# Autodesk Inventor assembly: ASY ДМФ 0100 Барабан v2.1
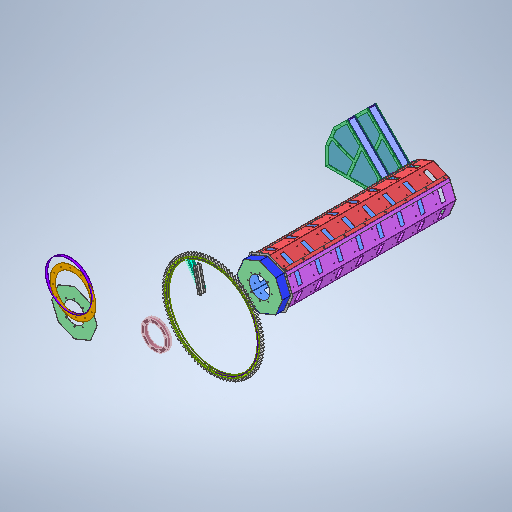
[picture p0: Inventor's stored thumbnail of the model, 512x512]
Saved by Autodesk Inventor 2025 (Build 290162010, 162A)
## iProperties
Created: 2024-04-28
Part Number: ASY ДМФ 0100 Барабан v2.1
Document SubType Name: Assembly
Designer: pokla
Author: pokla
## Documents named in this file (25)
- C:\Users\pokla\Documents\Inventor\ДФО\ДМФ\DMF-Disk-Micro-Filter\Барабан v2.1\ASY ДМФ 0100 Барабан v2.1.iam
- C:\Users\pokla\Documents\Inventor\ДФО\ДМФ\DMF-Disk-Micro-Filter\Барабан v2.1\DMF 01 21 Барабан торец НОС v2.1.ipt
- C:\Users\pokla\Documents\Inventor\ДФО\ДМФ\DMF-Disk-Micro-Filter\Барабан v2.1\DMF 01 13 Барабан Лист лев брт v2.1.ipt
- C:\Users\pokla\Documents\Inventor\ДФО\ДМФ\DMF-Disk-Micro-Filter\Барабан v2.1\DMF 01 14 Барабан Лист прав брт v2.1.ipt
- C:\Users\pokla\Documents\Inventor\ДФО\ДМФ\DMF-Disk-Micro-Filter\Барабан v2.1\DMF 01 31 Барабан Опорное кольцо НОС v2.1.ipt
- C:\Users\pokla\Documents\Inventor\ДФО\ДМФ\DMF-Disk-Micro-Filter\Барабан v2.1\DMF 01 17 опора крышки v2.1.ipt
- C:\Users\pokla\Documents\Inventor\ДФО\ДМФ\DMF-Disk-Micro-Filter\Барабан v2.1\DMF 000 размеры v2.1.ipt
- C:\Users\pokla\Documents\Inventor\ДФО\ДМФ\DMF-Disk-Micro-Filter\Барабан v2.1\DMF 01 12 Барабан усилитель v2.1.ipt
- C:\Users\pokla\Documents\Inventor\ДФО\ДМФ\DMF-Disk-Micro-Filter\Барабан v2.1\ASY DMF 010 cap v2.1.iam
- C:\Users\pokla\Documents\Inventor\ДФО\ДМФ\DMF-Disk-Micro-Filter\Барабан v2.1\DMF 01 32 Барабан Опорное кольцо КОРМА v2.1.ipt
- C:\Users\pokla\Documents\Inventor\ДФО\ДМФ\DMF-Disk-Micro-Filter\Барабан v2.1\DMF 01 22 Барабан торец КОРМА v2.1.ipt
- C:\Users\pokla\Documents\Inventor\ДФО\ДМФ\DMF-Disk-Micro-Filter\Барабан v2.1\ASY DMF filter package v2.1.iam
- C:\Users\pokla\Documents\Inventor\ДФО\ДМФ\DMF-Disk-Micro-Filter\Барабан v2.1\DMF 01 21 cylinder butt end nose.ipt
- C:\Users\pokla\Documents\Inventor\ДФО\ДМФ\DMF-Disk-Micro-Filter\Барабан v2.1\DMF 2.1 01 42 Gear way 2.ipt
- C:\Users\pokla\Documents\Inventor\ДФО\ДМФ\DMF-Disk-Micro-Filter\Барабан v2.1\DMF 2.1 01 43 Gear rim 3.ipt
- C:\Users\pokla\Documents\Inventor\ДФО\ДМФ\DMF-Disk-Micro-Filter\Барабан v2.1\DMF 2.1 01 44 Gear rim 4.ipt
- C:\Users\pokla\Documents\Inventor\ДФО\ДМФ\DMF-Disk-Micro-Filter\Барабан v2.1\DMF 2.1 01 45 Gear ring 5.ipt
- C:\Users\pokla\Documents\Inventor\ДФО\ДМФ\DMF-Disk-Micro-Filter\Барабан v2.1\DMF 2.1 01 46 Gear axis wheel 6.ipt
- C:\Users\pokla\Documents\Inventor\ДФО\ДМФ\DMF-Disk-Micro-Filter\Барабан v2.1\DMF 01 13 Барабан усилитель v2.1.ipt
- C:\Users\pokla\Documents\Inventor\ДФО\ДМФ\DMF-Disk-Micro-Filter\шестерни 06.09.2025\DMF sector big gear 2.1.ipt
- C:\Users\pokla\Documents\Inventor\ДФО\ДМФ\DMF-Disk-Micro-Filter\Барабан v2.1\DMF 01 15 drum sheet 1.ipt
- C:\Users\pokla\Documents\Inventor\ДФО\ДМФ\DMF-Disk-Micro-Filter\ДМФ 01 12 Барабан усилитель.ipt
- C:\Users\pokla\Documents\Inventor\ДФО\ДМФ\DMF-Disk-Micro-Filter\ДМФ 01 15 Барабан усилитель борта.ipt
- C:\Users\pokla\Documents\Inventor\ДФО\ДМФ\DMF-Disk-Micro-Filter\Барабан v2.1\DMF 2.1 Пластина паза маленькая.ipt
- C:\Users\pokla\Documents\Inventor\ДФО\ДМФ\DMF-Disk-Micro-Filter\Барабан v2.1\DMF 2.1 Пластина паза большая.ipt
## Components (92 placed, 25 different names)
1. DMF 000 размеры v2.1.ipt:1
2. DMF 01 21 Барабан торец НОС v2.1.ipt:1 — Mate:41, Flush:29, Flush:30, Mate:42, Flush:31, Flush:32
3. DMF 01 31 Барабан Опорное кольцо НОС v2.1.ipt:1
4. DMF 01 32 Барабан Опорное кольцо КОРМА v2.1.ipt:1 — Rigid:20
5. DMF 01 22 Барабан торец КОРМА v2.1.ipt:1 — Rigid:20, Rigid:51, Rigid:53, Mate:36, Flush:22, Flush:23, Mate:37, Flush:24, Flush:25, Mate:45, Flush:34, Flush:35
6. DMF 01 13 Барабан Лист лев брт v2.1.ipt:1 — Rigid:51
7. DMF 01 14 Барабан Лист прав брт v2.1.ipt:1 — Rigid:53, Rigid:60, Rigid:61
8. DMF 01 17 опора крышки v2.1.ipt:1 — Mate:37, Flush:24, Flush:25
9. DMF 01 17 опора крышки v2.1.ipt:2 — Mate:36, Flush:22, Flush:23
10. ASY DMF 010 cap v2.1.iam:1 [sub-assembly] — Mate:45, Flush:34, Flush:35, Flush:36, Mate:46, Mate:47
11. DMF 01 21 cylinder butt end nose.ipt:1
12. DMF 2.1 01 45 Gear ring 5.ipt:1
13. DMF 2.1 01 46 Gear axis wheel 6.ipt:1
14. DMF 2.1 01 44 Gear rim 4.ipt:1 — Rigid:39, Rigid:40, Rigid:41
15. DMF 2.1 01 43 Gear rim 3.ipt:2 — Rigid:24, Rigid:35
16. DMF 2.1 01 43 Gear rim 3.ipt:1 — Rigid:24
17. DMF 2.1 01 43 Gear rim 3.ipt:3 — Rigid:35, Rigid:36, Rigid:39
18. DMF 2.1 01 43 Gear rim 3.ipt:4
19. DMF 2.1 01 43 Gear rim 3.ipt:5 — Rigid:36, Rigid:38, Flush:18, Mate:33, Mate:34, Tangent:1
20. DMF 2.1 01 43 Gear rim 3.ipt:6 — Rigid:42
21. DMF 2.1 01 43 Gear rim 3.ipt:7 — Rigid:38
22. DMF 2.1 01 43 Gear rim 3.ipt:8
23. DMF 2.1 01 44 Gear rim 4.ipt:2 — Rigid:40
24. DMF 2.1 01 44 Gear rim 4.ipt:3 — Rigid:41
25. DMF 01 13 Барабан усилитель v2.1.ipt:2 — Rigid:43
26. DMF 01 12 Барабан усилитель v2.1.ipt:2 — Flush:18, Mate:33, Mate:34, Rigid:43, Flush:20
27. DMF 01 13 Барабан усилитель v2.1.ipt:1 — Tangent:1
28. DMF 01 12 Барабан усилитель v2.1.ipt:1 — Flush:20
29. DMF 01 15 drum sheet 1.ipt:1 — Mate:41, Flush:29, Flush:30, Flush:33, Mate:43
30. DMF 01 15 drum sheet 1.ipt:2 — Mate:42, Flush:31, Flush:32, Mate:44
31. ДМФ 01 12 Барабан усилитель.ipt:1 — Rigid:54, Rigid:55, Flush:36, Mate:46, Mate:47, Rigid:58
32. ДМФ 01 15 Барабан усилитель борта.ipt:1 — Rigid:54
33. ДМФ 01 15 Барабан усилитель борта.ipt:2 — Rigid:55
34. ДМФ 01 12 Барабан усилитель.ipt:2 — Rigid:56, Rigid:57, Flush:33, Mate:43, Mate:44, Rigid:58
35. ДМФ 01 15 Барабан усилитель борта.ipt:3 — Rigid:56
36. ДМФ 01 15 Барабан усилитель борта.ipt:4 — Rigid:57
37. DMF sector big gear 2.1.ipt:1 — Rigid:42
38. DMF sector big gear 2.1.ipt:2
39. DMF sector big gear 2.1.ipt:3
40. DMF sector big gear 2.1.ipt:4
41. DMF sector big gear 2.1.ipt:5
42. DMF sector big gear 2.1.ipt:6
43. DMF sector big gear 2.1.ipt:7
44. DMF sector big gear 2.1.ipt:8
45. DMF sector big gear 2.1.ipt:9
46. DMF sector big gear 2.1.ipt:10
47. DMF sector big gear 2.1.ipt:11
48. DMF sector big gear 2.1.ipt:12
49. DMF sector big gear 2.1.ipt:13
50. DMF sector big gear 2.1.ipt:14
51. DMF sector big gear 2.1.ipt:15
52. DMF sector big gear 2.1.ipt:16
53. DMF sector big gear 2.1.ipt:17
54. DMF sector big gear 2.1.ipt:18
55. DMF sector big gear 2.1.ipt:19
56. DMF sector big gear 2.1.ipt:20
57. DMF sector big gear 2.1.ipt:21
58. DMF sector big gear 2.1.ipt:22
59. DMF sector big gear 2.1.ipt:23
60. DMF sector big gear 2.1.ipt:24
61. DMF sector big gear 2.1.ipt:25
62. DMF sector big gear 2.1.ipt:26
63. DMF sector big gear 2.1.ipt:27
64. DMF sector big gear 2.1.ipt:28
65. DMF sector big gear 2.1.ipt:29
66. DMF sector big gear 2.1.ipt:30
67. DMF sector big gear 2.1.ipt:31
68. DMF sector big gear 2.1.ipt:32
69. DMF sector big gear 2.1.ipt:33
70. DMF sector big gear 2.1.ipt:34
71. DMF sector big gear 2.1.ipt:35
72. DMF sector big gear 2.1.ipt:36
73. DMF sector big gear 2.1.ipt:37
74. DMF sector big gear 2.1.ipt:38
75. DMF sector big gear 2.1.ipt:39
76. DMF sector big gear 2.1.ipt:40
77. DMF sector big gear 2.1.ipt:41
78. DMF sector big gear 2.1.ipt:42
79. DMF sector big gear 2.1.ipt:43
80. DMF sector big gear 2.1.ipt:44
81. DMF sector big gear 2.1.ipt:45
82. DMF sector big gear 2.1.ipt:46
83. DMF sector big gear 2.1.ipt:47
84. DMF sector big gear 2.1.ipt:48
85. DMF 2.1 01 42 Gear way 2.ipt:1 — Rigid:59, Rigid:60
86. ASY DMF filter package v2.1.iam:1 [sub-assembly] — Rigid:59
87. DMF 2.1 01 42 Gear way 2.ipt:2
88. ASY DMF filter package v2.1.iam:2 [sub-assembly]
89. DMF 2.1 Пластина паза большая:1 — Rigid:62
90. DMF 2.1 Пластина паза маленькая.ipt:1 — Rigid:61, Rigid:62
91. DMF 2.1 Пластина паза большая:2
92. DMF 2.1 Пластина паза маленькая:2
## Component patterns: (48 elements, first: DMF sector big gear 2.1.ipt:1), (2 elements, first: DMF 2.1 01 42 Gear way 2.ipt:1 + ASY DMF filter package v2.1.iam:1), (2 elements, first: DMF 2.1 Пластина паза большая:1 + DMF 2.1 Пластина паза маленькая.ipt:1)
## Relationships (51: WeldJoint 25, Flush 14, Mate 11, Tangent 1)
- Rigid:20 [WeldJoint]: DMF 01 32 Барабан Опорное кольцо КОРМА v2.1.ipt:1 ↔ DMF 01 22 Барабан торец КОРМА v2.1.ipt:1
- Rigid:24 [WeldJoint] (25 mm): DMF 2.1 01 43 Gear rim 3.ipt:2 ↔ DMF 2.1 01 43 Gear rim 3.ipt:1
- [WeldJoint] (25 mm): DMF 2.1 01 43 Gear rim 3.ipt:3 ↔ DMF 2.1 01 43 Gear rim 3.ipt:4
- [WeldJoint] (25 mm): DMF 2.1 01 43 Gear rim 3.ipt:5 ↔ DMF 2.1 01 43 Gear rim 3.ipt:6
- Rigid:35 [WeldJoint]: DMF 2.1 01 43 Gear rim 3.ipt:2 ↔ DMF 2.1 01 43 Gear rim 3.ipt:3
- Rigid:36 [WeldJoint]: DMF 2.1 01 43 Gear rim 3.ipt:3 ↔ DMF 2.1 01 43 Gear rim 3.ipt:5
- [WeldJoint] (25 mm): DMF 2.1 01 43 Gear rim 3.ipt:7 ↔ DMF 2.1 01 43 Gear rim 3.ipt:8
- Rigid:38 [WeldJoint]: DMF 2.1 01 43 Gear rim 3.ipt:5 ↔ DMF 2.1 01 43 Gear rim 3.ipt:7
- Rigid:39 [WeldJoint]: DMF 2.1 01 44 Gear rim 4.ipt:1 ↔ DMF 2.1 01 43 Gear rim 3.ipt:3
- Rigid:40 [WeldJoint]: DMF 2.1 01 44 Gear rim 4.ipt:1 ↔ DMF 2.1 01 44 Gear rim 4.ipt:2
- Rigid:41 [WeldJoint]: DMF 2.1 01 44 Gear rim 4.ipt:1 ↔ DMF 2.1 01 44 Gear rim 4.ipt:3
- Rigid:42 [WeldJoint]: DMF 2.1 01 43 Gear rim 3.ipt:6 ↔ DMF sector big gear 2.1.ipt:1
- Flush:18: DMF 2.1 01 43 Gear rim 3.ipt:5 ↔ DMF 01 12 Барабан усилитель v2.1.ipt:2
- Mate:33: DMF 2.1 01 43 Gear rim 3.ipt:5 ↔ DMF 01 12 Барабан усилитель v2.1.ipt:2
- Mate:34: DMF 2.1 01 43 Gear rim 3.ipt:5 ↔ DMF 01 12 Барабан усилитель v2.1.ipt:2
- Rigid:43 [WeldJoint]: DMF 01 13 Барабан усилитель v2.1.ipt:2 ↔ DMF 01 12 Барабан усилитель v2.1.ipt:2
- [WeldJoint]: DMF 01 13 Барабан усилитель v2.1.ipt:1 ↔ DMF 01 12 Барабан усилитель v2.1.ipt:1
- Flush:20: DMF 01 12 Барабан усилитель v2.1.ipt:2 ↔ DMF 01 12 Барабан усилитель v2.1.ipt:1
- Tangent:1: DMF 2.1 01 43 Gear rim 3.ipt:5 ↔ DMF 01 13 Барабан усилитель v2.1.ipt:1
- Rigid:51 [WeldJoint]: DMF 01 22 Барабан торец КОРМА v2.1.ipt:1 ↔ DMF 01 13 Барабан Лист лев брт v2.1.ipt:1
- Rigid:53 [WeldJoint]: DMF 01 22 Барабан торец КОРМА v2.1.ipt:1 ↔ DMF 01 14 Барабан Лист прав брт v2.1.ipt:1
- Mate:36: DMF 01 22 Барабан торец КОРМА v2.1.ipt:1 ↔ DMF 01 17 опора крышки v2.1.ipt:2
- Flush:22 (2 mm): DMF 01 22 Барабан торец КОРМА v2.1.ipt:1 ↔ DMF 01 17 опора крышки v2.1.ipt:2
- Flush:23 (2 mm): DMF 01 22 Барабан торец КОРМА v2.1.ipt:1 ↔ DMF 01 17 опора крышки v2.1.ipt:2
- Mate:37: DMF 01 22 Барабан торец КОРМА v2.1.ipt:1 ↔ DMF 01 17 опора крышки v2.1.ipt:1
- Flush:24 (2 mm): DMF 01 22 Барабан торец КОРМА v2.1.ipt:1 ↔ DMF 01 17 опора крышки v2.1.ipt:1
- Flush:25 (2 mm): DMF 01 22 Барабан торец КОРМА v2.1.ipt:1 ↔ DMF 01 17 опора крышки v2.1.ipt:1
- Rigid:54 [WeldJoint]: ДМФ 01 12 Барабан усилитель.ipt:1 ↔ ДМФ 01 15 Барабан усилитель борта.ipt:1
- Rigid:55 [WeldJoint]: ДМФ 01 12 Барабан усилитель.ipt:1 ↔ ДМФ 01 15 Барабан усилитель борта.ipt:2
- Rigid:56 [WeldJoint]: ДМФ 01 12 Барабан усилитель.ipt:2 ↔ ДМФ 01 15 Барабан усилитель борта.ipt:3
- Rigid:57 [WeldJoint]: ДМФ 01 12 Барабан усилитель.ipt:2 ↔ ДМФ 01 15 Барабан усилитель борта.ipt:4
- Mate:41: DMF 01 21 Барабан торец НОС v2.1.ipt:1 ↔ DMF 01 15 drum sheet 1.ipt:1
- Flush:29: DMF 01 21 Барабан торец НОС v2.1.ipt:1 ↔ DMF 01 15 drum sheet 1.ipt:1
- Flush:30: DMF 01 21 Барабан торец НОС v2.1.ipt:1 ↔ DMF 01 15 drum sheet 1.ipt:1
- Mate:42: DMF 01 21 Барабан торец НОС v2.1.ipt:1 ↔ DMF 01 15 drum sheet 1.ipt:2
- Flush:31: DMF 01 21 Барабан торец НОС v2.1.ipt:1 ↔ DMF 01 15 drum sheet 1.ipt:2
- Flush:32: DMF 01 21 Барабан торец НОС v2.1.ipt:1 ↔ DMF 01 15 drum sheet 1.ipt:2
- Flush:33: DMF 01 15 drum sheet 1.ipt:1 ↔ ДМФ 01 12 Барабан усилитель.ipt:2
- Mate:43: DMF 01 15 drum sheet 1.ipt:1 ↔ ДМФ 01 12 Барабан усилитель.ipt:2
- Mate:44: DMF 01 15 drum sheet 1.ipt:2 ↔ ДМФ 01 12 Барабан усилитель.ipt:2
- Mate:45: DMF 01 22 Барабан торец КОРМА v2.1.ipt:1 ↔ ASY DMF 010 cap v2.1.iam:1
- Flush:34: DMF 01 22 Барабан торец КОРМА v2.1.ipt:1 ↔ ASY DMF 010 cap v2.1.iam:1
- Flush:35: DMF 01 22 Барабан торец КОРМА v2.1.ipt:1 ↔ ASY DMF 010 cap v2.1.iam:1
- Flush:36: ASY DMF 010 cap v2.1.iam:1 ↔ ДМФ 01 12 Барабан усилитель.ipt:1
- Mate:46: ASY DMF 010 cap v2.1.iam:1 ↔ ДМФ 01 12 Барабан усилитель.ipt:1
- Mate:47: ASY DMF 010 cap v2.1.iam:1 ↔ ДМФ 01 12 Барабан усилитель.ipt:1
- Rigid:58 [WeldJoint]: ДМФ 01 12 Барабан усилитель.ipt:1 ↔ ДМФ 01 12 Барабан усилитель.ipt:2
- Rigid:59 [WeldJoint] (5 mm): DMF 2.1 01 42 Gear way 2.ipt:1 ↔ ASY DMF filter package v2.1.iam:1
- Rigid:60 [WeldJoint]: DMF 01 14 Барабан Лист прав брт v2.1.ipt:1 ↔ DMF 2.1 01 42 Gear way 2.ipt:1
- Rigid:61 [WeldJoint] (-48.5 mm): DMF 01 14 Барабан Лист прав брт v2.1.ipt:1 ↔ DMF 2.1 Пластина паза маленькая.ipt:1
- Rigid:62 [WeldJoint]: DMF 2.1 Пластина паза большая:1 ↔ DMF 2.1 Пластина паза маленькая.ipt:1
## Named parameters: d314_d251 = 25 mm, d315_d251 = 25 mm, d318_d251 = 25 mm, d336_d335 = 0 mm
